# Autodesk Inventor assembly: WHEEL X SHAFT
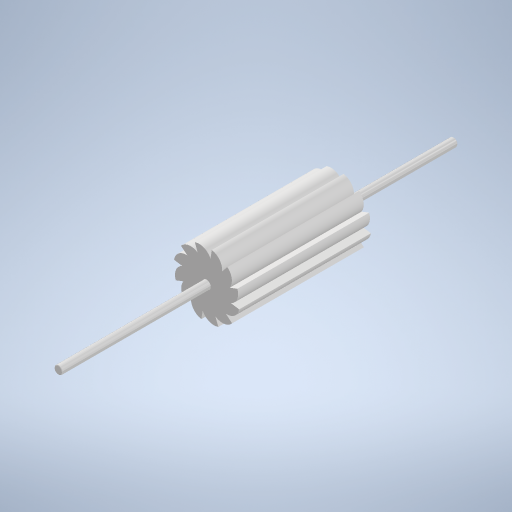
[picture p0: Inventor's stored thumbnail of the model, 512x512]
Saved by Autodesk Inventor 2023 (Build 270158000, 158)
## iProperties
Created: 2023-01-29
Part Number: WHEEL X SHAFT
Document SubType Name: Assembly
Designer: Steven
Author: Steven
## Documents named in this file (3)
- C:\Users\steve\OneDrive\Documents\McMaster University\Courses-Year5\4TB6 Capstone Design Project\The_Nursery_Project\parts\Tray Dropper\ALTERNATIVE SOLUTION\WHEEL X SHAFT.iam
- C:\Users\steve\OneDrive\Documents\McMaster University\Courses-Year5\4TB6 Capstone Design Project\The_Nursery_Project\parts\Tray Dropper\ALTERNATIVE SOLUTION\THE_WHEEL 2.0.ipt
- C:\Users\steve\Downloads\8632T139_D-Profile Rotary Shaft.ipt
## Components (2 placed, 2 different names)
1. THE_WHEEL 2.0:1 — Mate:1, Mate:2, Flush:1
2. 8632T139_D-Profile Rotary Shaft:1 — Mate:1, Mate:2, Mate:4, Flush:1
## Relationships (4: Mate 3, Flush 1)
- Mate:1: THE_WHEEL 2.0:1 ↔ 8632T139_D-Profile Rotary Shaft:1
- Mate:2: THE_WHEEL 2.0:1 ↔ 8632T139_D-Profile Rotary Shaft:1
- Mate:4: 8632T139_D-Profile Rotary Shaft:1
- Flush:1 (114.3 mm): THE_WHEEL 2.0:1 ↔ 8632T139_D-Profile Rotary Shaft:1
